# Autodesk Inventor assembly: Eje-engrane
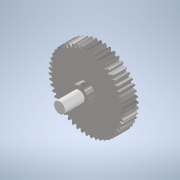
[picture p0: Inventor's stored thumbnail of the model, 180x180]
Saved by Autodesk Inventor 2021 (Build 250183000, 183)
## iProperties
Created: 2021-02-07
Part Number: Eje-engrane
Document SubType Name: Assembly
Designer: rotje
Author: rotje
## Documents named in this file (3)
- C:\Users\rotje\Documents\Inventor\MSF\Eje-engrane.iam
- C:\Users\rotje\Documents\Inventor\MSF\Engranaje recto_50_Dientes.ipt
- C:\Users\rotje\Documents\Inventor\MSF\Eje_engrane.ipt
## Components (2 placed, 2 different names)
1. Engranaje recto2:1 — Insertar:1
2. Eje_engrane:1 — Insertar:1
## Relationships (1: Insert 1)
- Insertar:1 (10 mm): Engranaje recto2:1 ↔ Eje_engrane:1
